# Autodesk Inventor assembly: RailAndMirror
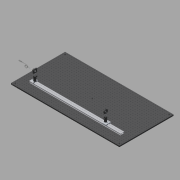
[picture p0: Inventor's stored thumbnail of the model, 180x180]
Saved by Autodesk Inventor 2018 (Build 220112000, 112)
## iProperties
Created: 2018-09-17
Part Number: RailAndMirror
Document SubType Name: Assembly
Designer: Robert Campbell
Author: Robert Campbell
## Documents named in this file (9)
- \\Mac\Home\Dropbox (UCL - SWC)\work\WorkDocs\MF_BenchOptics\CAD_files\RailAndMirror.iam
- \\Mac\Home\Dropbox (UCL - SWC)\work\WorkDocs\MF_BenchOptics\CAD_files\MB60120_M-Solidworks.ipt
- \\Mac\Home\Dropbox (UCL - SWC)\work\WorkDocs\MF_BenchOptics\CAD_files\XT66DP-1000-Solidworks.ipt
- \\Mac\Home\Dropbox (UCL - SWC)\work\WorkDocs\MF_BenchOptics\CAD_files\KAD11F-Solidworks.ipt
- \\Mac\Home\Dropbox (UCL - SWC)\work\WorkDocs\MF_BenchOptics\CAD_files\CPS635R-Solidworks.ipt
- \\Mac\Home\Dropbox (UCL - SWC)\work\WorkDocs\MF_BenchOptics\CAD_files\CP02_M-Solidworks.ipt
- \\Mac\Home\Dropbox (UCL - SWC)\work\WorkDocs\MF_BenchOptics\CAD_files\PH50_and_carriage.iam
- \\Mac\Home\Dropbox (UCL - SWC)\work\WorkDocs\MF_BenchOptics\CAD_files\TR50_M-Solidworks.ipt
- \\Mac\Home\Dropbox (UCL - SWC)\work\WorkDocs\MF_BenchOptics\CAD_files\ID25_M-Solidworks.ipt
## Components (9 placed, 8 different names)
1. MB60120_M-Solidworks:1 — Mate:1
2. XT66DP-1000-Solidworks:1 — Mate:1, Mate:9, Mate:10, Mate:13, Angle:3
3. KAD11F-Solidworks:1 — Mate:2, Flush:1, Mate:4
4. CPS635R-Solidworks:1 — Mate:2, Flush:1, Mate:3
5. CP02_M-Solidworks:1 — Mate:3, Mate:4, Mate:5, Mate:6, Angle:1
6. PH50_and_carriage:1 [sub-assembly] — Mate:7, Mate:8, Angle:1, Mate:9, Mate:10
7. TR50_M-Solidworks:1 — Mate:5, Mate:6, Mate:7, Mate:8
8. ID25_M-Solidworks:1 — Mate:11, Mate:12, Angle:2
9. PH50_and_carriage:2 [sub-assembly] — Mate:11, Mate:12, Angle:2, Mate:13, Angle:3
## Relationships (17: Mate 13, Angle 3, Flush 1)
- Mate:1: MB60120_M-Solidworks:1 ↔ XT66DP-1000-Solidworks:1
- Mate:2: KAD11F-Solidworks:1 ↔ CPS635R-Solidworks:1
- Flush:1 (-5 mm): KAD11F-Solidworks:1 ↔ CPS635R-Solidworks:1
- Mate:3: CPS635R-Solidworks:1 ↔ CP02_M-Solidworks:1
- Mate:4: KAD11F-Solidworks:1 ↔ CP02_M-Solidworks:1
- Mate:5: CP02_M-Solidworks:1 ↔ TR50_M-Solidworks:1
- Mate:6: CP02_M-Solidworks:1 ↔ TR50_M-Solidworks:1
- Mate:7: PH50_and_carriage:1 ↔ TR50_M-Solidworks:1
- Mate:8 (20 mm): PH50_and_carriage:1 ↔ TR50_M-Solidworks:1
- Angle:1 (0 deg): CP02_M-Solidworks:1 ↔ PH50_and_carriage:1
- Mate:9: XT66DP-1000-Solidworks:1 ↔ PH50_and_carriage:1
- Mate:10 (-40 mm): XT66DP-1000-Solidworks:1 ↔ PH50_and_carriage:1
- Mate:11: ID25_M-Solidworks:1 ↔ PH50_and_carriage:2
- Mate:12 (26 mm): ID25_M-Solidworks:1 ↔ PH50_and_carriage:2
- Angle:2 (0 deg): ID25_M-Solidworks:1 ↔ PH50_and_carriage:2
- Mate:13: XT66DP-1000-Solidworks:1 ↔ PH50_and_carriage:2
- Angle:3 (0 deg): XT66DP-1000-Solidworks:1 ↔ PH50_and_carriage:2
